# Autodesk Inventor assembly: standard_assy
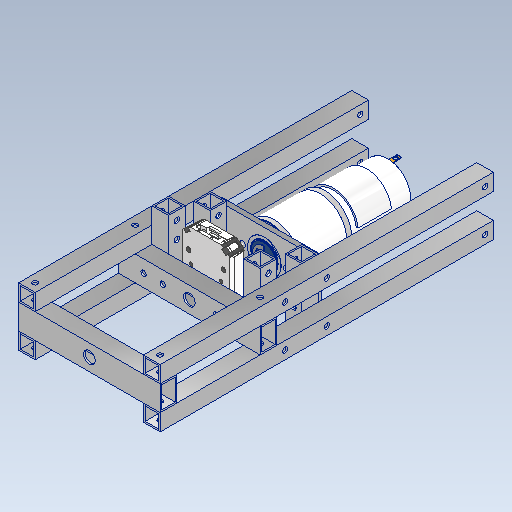
[picture p0: Inventor's stored thumbnail of the model, 512x512]
Saved by Autodesk Inventor 2027.1 (Build 311270010, 270A)
## iProperties
Created: 2026-10-09
Part Number: standard_assy
Document SubType Name: Assembly
Designer: ug_nd
Author: ug_nd
## Documents named in this file (9)
- C:\Users\ug_nd\git_local\3wd_mecanums\cad\standard_assy\standard_assy.iam
- C:\Users\ug_nd\git_local\3wd_mecanums\cad\standard_assy\alsp_10_15_85_1.ipt
- C:\Users\ug_nd\git_local\3wd_mecanums\cad\common_parts\Geared_RS-385\Geared_RS-385.iam
- C:\Users\ug_nd\git_local\3wd_mecanums\cad\standard_assy\alsp_10_10_45_1.ipt
- C:\Users\ug_nd\git_local\3wd_mecanums\cad\standard_assy\alsp_10_10_200_1.ipt
- C:\Users\ug_nd\git_local\3wd_mecanums\cad\standard_assy\alsp_10_15_85_2.ipt
- C:\Users\ug_nd\git_local\3wd_mecanums\cad\standard_assy\alsp_10_10_35_1.ipt
- C:\Users\ug_nd\git_local\3wd_mecanums\cad\standard_assy\alfs_3_63_30_1.ipt
- C:\Users\ug_nd\git_local\3wd_mecanums\cad\common_parts\amt102-v\amt102-v.iam
## Components (13 placed, 8 different names)
1. alsp_10_15_85_1:1 — メイト:1, フラッシュ:1, フラッシュ:2, メイト:3, メイト:4, メイト:7, メイト:9, メイト:11, メイト:13, メイト:30, メイト:31, メイト:32, メイト:33, メイト:34
2. alsp_10_10_200_1:1 — メイト:7, メイト:8, メイト:15, メイト:17, メイト:18, メイト:20
3. alsp_10_10_200_1:2 — メイト:9, メイト:10, メイト:19
4. alsp_10_10_200_1:3 — メイト:11, メイト:12, メイト:16, メイト:21, メイト:23
5. alsp_10_10_200_1:4 — メイト:13, メイト:14, メイト:22
6. alsp_10_10_45_1:1 — メイト:3, メイト:8, メイト:10
7. alsp_10_10_45_1:2 — メイト:4, メイト:12, メイト:14
8. alsp_10_10_35_1:1 — メイト:18, メイト:19, メイト:20, メイト:27, メイト:29
9. alsp_10_10_35_1:2 — メイト:21, メイト:22, メイト:23, メイト:28
10. alfs_3_63_30_1:1 — メイト:24, メイト:25, メイト:26, メイト:27, メイト:28, メイト:29
11. Geared_RS-385:1 [sub-assembly] — メイト:2, メイト:24, メイト:25, メイト:26
12. alsp_10_15_85_2:1 — メイト:15, メイト:16, メイト:17
13. amt102-v:1 [sub-assembly] — メイト:30, メイト:31, メイト:32, メイト:33, メイト:34
## Relationships (34: Mate 32, Flush 2)
- メイト:1 [Mate]: alsp_10_15_85_1:1
- フラッシュ:1 [Flush]: alsp_10_15_85_1:1
- フラッシュ:2 [Flush]: alsp_10_15_85_1:1
- メイト:2 [Mate]: Geared_RS-385:1
- メイト:3 [Mate]: alsp_10_15_85_1:1 ↔ alsp_10_10_45_1:1
- メイト:4 [Mate]: alsp_10_15_85_1:1 ↔ alsp_10_10_45_1:2
- メイト:7 [Mate]: alsp_10_15_85_1:1 ↔ alsp_10_10_200_1:1
- メイト:8 [Mate]: alsp_10_10_200_1:1 ↔ alsp_10_10_45_1:1
- メイト:9 [Mate]: alsp_10_15_85_1:1 ↔ alsp_10_10_200_1:2
- メイト:10 [Mate]: alsp_10_10_200_1:2 ↔ alsp_10_10_45_1:1
- メイト:11 [Mate]: alsp_10_15_85_1:1 ↔ alsp_10_10_200_1:3
- メイト:12 [Mate]: alsp_10_10_200_1:3 ↔ alsp_10_10_45_1:2
- メイト:13 [Mate]: alsp_10_15_85_1:1 ↔ alsp_10_10_200_1:4
- メイト:14 [Mate]: alsp_10_10_200_1:4 ↔ alsp_10_10_45_1:2
- メイト:15 [Mate]: alsp_10_10_200_1:1 ↔ alsp_10_15_85_2:1
- メイト:16 [Mate]: alsp_10_10_200_1:3 ↔ alsp_10_15_85_2:1
- メイト:17 [Mate]: alsp_10_10_200_1:1 ↔ alsp_10_15_85_2:1
- メイト:18 [Mate]: alsp_10_10_200_1:1 ↔ alsp_10_10_35_1:1
- メイト:19 [Mate]: alsp_10_10_200_1:2 ↔ alsp_10_10_35_1:1
- メイト:20 [Mate]: alsp_10_10_200_1:1 ↔ alsp_10_10_35_1:1
- メイト:21 [Mate]: alsp_10_10_200_1:3 ↔ alsp_10_10_35_1:2
- メイト:22 [Mate]: alsp_10_10_200_1:4 ↔ alsp_10_10_35_1:2
- メイト:23 [Mate]: alsp_10_10_200_1:3 ↔ alsp_10_10_35_1:2
- メイト:24 [Mate]: alfs_3_63_30_1:1 ↔ Geared_RS-385:1
- メイト:25 [Mate]: alfs_3_63_30_1:1 ↔ Geared_RS-385:1
- メイト:26 [Mate]: alfs_3_63_30_1:1 ↔ Geared_RS-385:1
- メイト:27 [Mate]: alsp_10_10_35_1:1 ↔ alfs_3_63_30_1:1
- メイト:28 [Mate]: alsp_10_10_35_1:2 ↔ alfs_3_63_30_1:1
- メイト:29 [Mate]: alsp_10_10_35_1:1 ↔ alfs_3_63_30_1:1
- メイト:30 [Mate]: alsp_10_15_85_1:1 ↔ amt102-v:1
- メイト:31 [Mate]: alsp_10_15_85_1:1 ↔ amt102-v:1
- メイト:32 [Mate]: alsp_10_15_85_1:1 ↔ amt102-v:1
- メイト:33 [Mate]: alsp_10_15_85_1:1 ↔ amt102-v:1
- メイト:34 [Mate]: alsp_10_15_85_1:1 ↔ amt102-v:1
